# Autodesk Inventor assembly: Front Lead Screw Idler
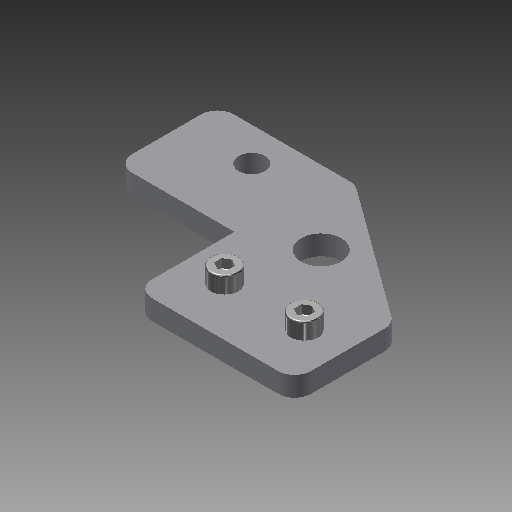
[picture p0: Inventor's stored thumbnail of the model, 512x512]
Saved by Autodesk Inventor 2017 (Build 210142000, 142)
## iProperties
Created: 2016-08-02
Part Number: Front Lead Screw Idler
Document SubType Name: Assembly
Designer: User
Author: User
## Documents named in this file (5)
- C:\All INVENTOR\SL-Inventor\SL-Beast 3D Printer\Front Lead Screw Idler.iam
- C:\All INVENTOR\SL-Inventor\SL-Beast 3D Printer\Leadscrew-rod-holder_MIR.ipt
- C:\All INVENTOR\SL-Inventor\SL-Beast 3D Printer\en-US\ANSI B18.3.1M(6)\ANSI B18.3.1M - M5x0.8 x 12(1).ipt
- C:\All INVENTOR\SL-Inventor\SL-Beast 3D Printer\M5 Tee Nut-Generic_MIR_MIR.ipt
- C:\All INVENTOR\SL-Inventor\SL-Beast 3D Printer\M5 Tee Nut-Generic_MIR_CPY_MIR.ipt
## Components (5 placed, 4 different names)
1. Leadscrew-rod-holder_MIR:1
2. Forged Socket Head Cap Screw - Metric M5x0.8 x 12:1
3. Forged Socket Head Cap Screw - Metric M5x0.8 x 12:2
4. M5 Tee Nut-Generic_MIR_MIR:1
5. M5 Tee Nut-Generic_MIR_CPY_MIR:1
## Relationships (7: Mate 6, Flush 1)
- [Mate]: Leadscrew-rod-holder_MIR:1 ↔ Forged Socket Head Cap Screw - Metric M5x0.8 x 12:1
- [Mate]: Leadscrew-rod-holder_MIR:1 ↔ Forged Socket Head Cap Screw - Metric M5x0.8 x 12:1
- [Mate]: Leadscrew-rod-holder_MIR:1 ↔ Forged Socket Head Cap Screw - Metric M5x0.8 x 12:2
- [Mate]: Leadscrew-rod-holder_MIR:1 ↔ Forged Socket Head Cap Screw - Metric M5x0.8 x 12:2
- [Mate]: Forged Socket Head Cap Screw - Metric M5x0.8 x 12:1 ↔ M5 Tee Nut-Generic_MIR_MIR:1
- [Flush]: M5 Tee Nut-Generic_MIR_MIR:1 ↔ M5 Tee Nut-Generic_MIR_CPY_MIR:1
- [Mate]: Forged Socket Head Cap Screw - Metric M5x0.8 x 12:2 ↔ M5 Tee Nut-Generic_MIR_CPY_MIR:1
